# Autodesk Inventor assembly: 麥克風組_MIR
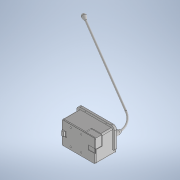
[picture p0: Inventor's stored thumbnail of the model, 180x180]
Saved by Autodesk Inventor 2021 (Build 250183000, 183)
## iProperties
Created: 2023-02-28
Part Number: 麥克風組_MIR
Document SubType Name: Assembly
Designer: brian
Author: brian
## Documents named in this file (3)
- C:\Users\brian\Desktop\自動主席台\麥克風組_MIR.iam
- C:\Users\brian\Desktop\自動主席台\麥克風崁座_MIR.ipt
- C:\Users\brian\Desktop\自動主席台\準確無線麥克風組_MIR.ipt
## Components (2 placed, 2 different names)
1. 麥克風崁座_MIR:1 — 貼合:1, 齊平:3, 齊平:2
2. 準確無線麥克風組_MIR:1 — 貼合:1, 齊平:3, 齊平:2
## Relationships (3: Flush 2, Mate 1)
- 貼合:1 [Mate]: 麥克風崁座_MIR:1 ↔ 準確無線麥克風組_MIR:1
- 齊平:3 [Flush]: 麥克風崁座_MIR:1 ↔ 準確無線麥克風組_MIR:1
- 齊平:2 [Flush]: 麥克風崁座_MIR:1 ↔ 準確無線麥克風組_MIR:1
